# Autodesk Inventor assembly: Motor
Saved by Autodesk Inventor 2014 SP1 (Build 180222100, 222)
## iProperties
Created: 2014-03-25
Part Number: Motor
Document SubType Name: Assembly
Designer: tom
Author: tom
## Documents named in this file (4)
- C:\Users\tom\Documents\GitHub\Boat_Bot\Motor.iam
- C:\Users\tom\Documents\GitHub\Boat_Bot\Part1.ipt
- C:\Users\tom\Documents\GitHub\Boat_Bot\Part2.ipt
- C:\Users\tom\Documents\GitHub\Boat_Bot\Part3.ipt
## Components (3 placed, 3 different names)
1. Part1:1
2. Part2:1
3. Part3:1
## Relationships (2: Flush 2)
- [Flush]: Part1:1 ↔ Part2:1
- [Flush]: Part2:1 ↔ Part3:1
